# Autodesk Inventor assembly: Хвост
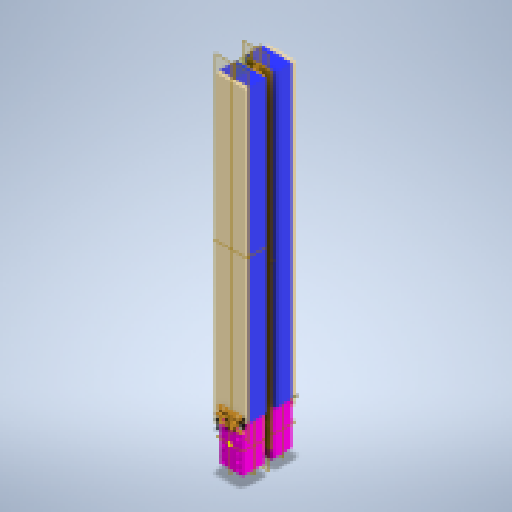
[picture p0: Inventor's stored thumbnail of the model, 512x512]
Saved by Autodesk Inventor 2023.2 (Build 272271030, 271C)
## iProperties
Created: 2024-03-12
Part Number: Хвост
Document SubType Name: Assembly
Designer: I9232
Author: I9232
## Documents named in this file (9)
- D:\!project\fox_n_crow_construction\crow\face\Хвост.iam
- D:\!project\fox_n_crow_construction\crow\face\Алюминиевый профиль.ipt
- D:\!project\fox_n_crow_construction\crow\face\Веер хвоста (сложенный).ipt
- D:\!project\fox_n_crow_construction\crow\face\Фанерка хвоста.ipt
- D:\!project\fox_n_crow_construction\crow\face\Петля.ipt
- D:\!project\fox_n_crow_construction\crow\face\крепление петли хвоста.ipt
- D:\!project\fox_n_crow_construction\crow\face\Веер хвоста (сложенный)_MIR.ipt
- D:\!project\fox_n_crow_construction\crow\face\Фанерка хвоста_MIR.ipt
- D:\!project\fox_n_crow_construction\crow\face\Петля_MIR.ipt
## Components (9 placed, 8 different names)
1. Алюминиевый профиль:1 — Совмещение:1, Совмещение:2, Совмещение:9, Совмещение:10, Совмещение:17, Совмещение:18, Совмещение:19, Совмещение:20
2. Веер хвоста (сложенный):1 — Совмещение:1, Совмещение:2, Совмещение:4, Совмещение:5, Совмещение:11
3. Фанерка хвоста:1 — Совмещение:4, Совмещение:5, Совмещение:6, Совмещение:7, Совмещение:8
4. Петля:1 — Совмещение:6, Совмещение:7, Совмещение:8
5. крепление петли хвоста:1 — Совмещение:9, Совмещение:10, Совмещение:11
6. Веер хвоста (сложенный)_MIR:1 — Совмещение:12, Совмещение:13, Совмещение:18, Совмещение:19, Совмещение:20
7. Фанерка хвоста_MIR:1 — Совмещение:12, Совмещение:13, Совмещение:14, Совмещение:15, Совмещение:16
8. Петля_MIR:1 — Совмещение:14, Совмещение:15, Совмещение:16, Совмещение:21, Совмещение:22
9. крепление петли хвоста:2 — Совмещение:17, Совмещение:21, Совмещение:22
## Relationships (21: Mate 21)
- Совмещение:1 [Mate]: Алюминиевый профиль:1 ↔ Веер хвоста (сложенный):1
- Совмещение:2 [Mate]: Алюминиевый профиль:1 ↔ Веер хвоста (сложенный):1
- Совмещение:4 [Mate]: Веер хвоста (сложенный):1 ↔ Фанерка хвоста:1
- Совмещение:5 [Mate]: Веер хвоста (сложенный):1 ↔ Фанерка хвоста:1
- Совмещение:6 [Mate]: Фанерка хвоста:1 ↔ Петля:1
- Совмещение:7 [Mate] (28.5 mm): Фанерка хвоста:1 ↔ Петля:1
- Совмещение:8 [Mate]: Фанерка хвоста:1 ↔ Петля:1
- Совмещение:9 [Mate]: Алюминиевый профиль:1 ↔ крепление петли хвоста:1
- Совмещение:10 [Mate]: Алюминиевый профиль:1 ↔ крепление петли хвоста:1
- Совмещение:11 [Mate]: Веер хвоста (сложенный):1 ↔ крепление петли хвоста:1
- Совмещение:12 [Mate]: Веер хвоста (сложенный)_MIR:1 ↔ Фанерка хвоста_MIR:1
- Совмещение:13 [Mate]: Веер хвоста (сложенный)_MIR:1 ↔ Фанерка хвоста_MIR:1
- Совмещение:14 [Mate]: Фанерка хвоста_MIR:1 ↔ Петля_MIR:1
- Совмещение:15 [Mate] (28.5 mm): Фанерка хвоста_MIR:1 ↔ Петля_MIR:1
- Совмещение:16 [Mate]: Фанерка хвоста_MIR:1 ↔ Петля_MIR:1
- Совмещение:17 [Mate]: Алюминиевый профиль:1 ↔ крепление петли хвоста:2
- Совмещение:18 [Mate]: Алюминиевый профиль:1 ↔ Веер хвоста (сложенный)_MIR:1
- Совмещение:19 [Mate]: Алюминиевый профиль:1 ↔ Веер хвоста (сложенный)_MIR:1
- Совмещение:20 [Mate]: Алюминиевый профиль:1 ↔ Веер хвоста (сложенный)_MIR:1
- Совмещение:21 [Mate]: Петля_MIR:1 ↔ крепление петли хвоста:2
- Совмещение:22 [Mate]: Петля_MIR:1 ↔ крепление петли хвоста:2
